# Autodesk Inventor assembly: Main
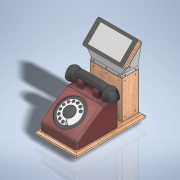
[picture p0: Inventor's stored thumbnail of the model, 180x180]
Saved by Autodesk Inventor 2020.2 (Build 242310000, 310)
## iProperties
Created: 2020-02-25
Part Number: Main
Document SubType Name: Assembly
Designer: sdekr
Author: sdekr
## Documents named in this file (8)
- D:\Inventor\Project PAD\Main.iam
- D:\Inventor\Project PAD\Phone\Phone_Complete.ipt
- D:\Inventor\Project PAD\Frame.iam
- D:\Inventor\Project PAD\LCD\Screen assembly.iam
- D:\Inventor\Project FYS\RQ-50B.ipt
- D:\Inventor\Project FYS\IEC320-C14.ipt
- D:\Inventor\Project PAD\Rpi3Bplus.ipt
- D:\Inventor\Project FYS\909.ipt
## Components (7 placed, 7 different names)
1. Phone_Complete:1 — Mate:1, Mate:2, Flush:4, Mate:9
2. Frame:1 [sub-assembly] — Mate:2, Flush:4, Mate:12, Mate:13, Mate:14, Mate:18, Mate:19, Mate:20, Mate:21, Mate:22, Mate:23, Mate:25, Flush:5, Tangent:1, Mate:26, Mate:27, Mate:28
3. Screen assembly:1 [sub-assembly] — Mate:9, Mate:26, Mate:27, Mate:28
4. RQ-50B:1 — Mate:12, Mate:13, Mate:14
5. Rpi3Bplus:1 — Mate:18, Mate:19, Mate:20
6. IEC320-C14:1 — Mate:21, Mate:22, Mate:23
7. 909:1 — Mate:25, Flush:5, Tangent:1
## Relationships (19: Mate 16, Flush 2, Tangent 1)
- Mate:1: Phone_Complete:1
- Mate:2: Phone_Complete:1 ↔ Frame:1
- Flush:4 (-10 mm): Phone_Complete:1 ↔ Frame:1
- Mate:9: Phone_Complete:1 ↔ Screen assembly:1
- Mate:12: Frame:1 ↔ RQ-50B:1
- Mate:13 (5 mm): Frame:1 ↔ RQ-50B:1
- Mate:14 (5 mm): Frame:1 ↔ RQ-50B:1
- Mate:18 (2 mm): Frame:1 ↔ Rpi3Bplus:1
- Mate:19: Frame:1 ↔ Rpi3Bplus:1
- Mate:20 (5 mm): Frame:1 ↔ Rpi3Bplus:1
- Mate:21: Frame:1 ↔ IEC320-C14:1
- Mate:22: Frame:1 ↔ IEC320-C14:1
- Mate:23: Frame:1 ↔ IEC320-C14:1
- Mate:25: Frame:1 ↔ 909:1
- Flush:5: Frame:1 ↔ 909:1
- Tangent:1: Frame:1 ↔ 909:1
- Mate:26: Frame:1 ↔ Screen assembly:1
- Mate:27: Frame:1 ↔ Screen assembly:1
- Mate:28: Frame:1 ↔ Screen assembly:1
